# Autodesk Inventor assembly: Assembly1
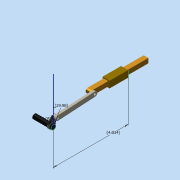
[picture p0: Inventor's stored thumbnail of the model, 180x180]
Saved by Autodesk Inventor 2017 (Build 210142000, 142)
## iProperties
Created: 2016-10-24
Part Number: Assembly1
Document SubType Name: Assembly
Designer: techn
Author: techn
## Documents named in this file (6)
- D:\OneDrive\Documents\Other Projects\Submarine\CAD\aft\Test\MotionTest\Assembly1.iam
- D:\OneDrive\Documents\Other Projects\Submarine\CAD\aft\Test\MotionTest\Part1.ipt
- D:\OneDrive\Documents\Other Projects\Submarine\CAD\aft\Test\MotionTest\Part2.ipt
- D:\OneDrive\Documents\Other Projects\Submarine\CAD\aft\Test\MotionTest\Part3.ipt
- D:\OneDrive\Documents\Other Projects\Submarine\CAD\aft\Test\MotionTest\Part4.ipt
- D:\OneDrive\Documents\Other Projects\Submarine\CAD\aft\Test\MotionTest\Part5.ipt
## Components (5 placed, 5 different names)
1. Part1:1 — Mate:1, Mate:2, Mate:3, Mate:4
2. Part2:1 — Mate:5, Mate:6, Mate:7
3. Part3:1 — Mate:3, Mate:4, Mate:5, Mate:6
4. Part4:1 — Mate:7, Flush:1
5. Part5:1 — Mate:1, Mate:2, Flush:1
## Relationships (8: Mate 7, Flush 1)
- Mate:1: Part1:1 ↔ Part5:1
- Mate:2: Part1:1 ↔ Part5:1
- Mate:3: Part1:1 ↔ Part3:1
- Mate:4: Part1:1 ↔ Part3:1
- Mate:5: Part2:1 ↔ Part3:1
- Mate:6: Part2:1 ↔ Part3:1
- Mate:7: Part2:1 ↔ Part4:1
- Flush:1: Part4:1 ↔ Part5:1
